# Autodesk Inventor assembly: 090 ASY bottom
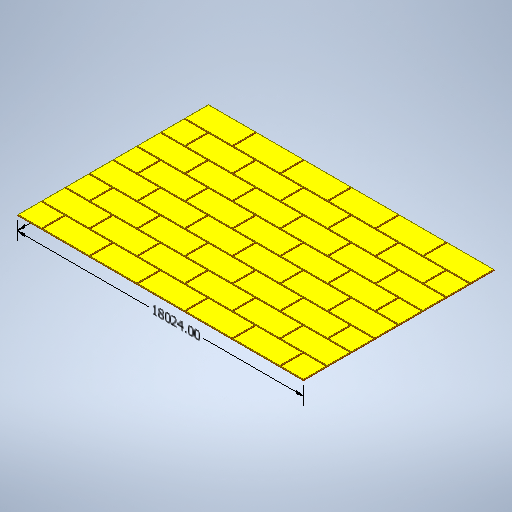
[picture p0: Inventor's stored thumbnail of the model, 512x512]
Saved by Autodesk Inventor 2026.2 (Build 302298000, 298)
## iProperties
Created: 2026-05-19
Part Number: 090 ASY bottom
Document SubType Name: Assembly
Designer: user
Author: user
## Documents named in this file (6)
- C:\Users\admin\Documents\Inventor\GBK-Gubkinskiy\090 ASY bottom.iam
- C:\Users\admin\Documents\Inventor\GBK-Gubkinskiy\0910.ipt
- C:\Users\admin\Documents\Inventor\GBK-Gubkinskiy\092_CPY.iam
- C:\Users\admin\Documents\Inventor\GBK-Gubkinskiy\093_CPY.iam
- C:\Users\admin\Documents\Inventor\GBK-Gubkinskiy\092_CPY1.iam
- C:\Users\admin\Documents\Inventor\GBK-Gubkinskiy\093_CPY1.iam
## Components (53 placed, 5 different names)
1. 0910:1 — Rigid:1
2. 093_CPY:1 [sub-assembly] — Flush:3, Flush:4, Mate:1, Flush:5, Flush:6, Mate:2
3. 093_CPY1:1 [sub-assembly] — Flush:7, Flush:8, Mate:3
4. 093_CPY:2 [sub-assembly]
5. 093_CPY1:2 [sub-assembly]
6. 093_CPY:3 [sub-assembly]
7. 093_CPY1:3 [sub-assembly]
8. 093_CPY:4 [sub-assembly]
9. 093_CPY1:4 [sub-assembly]
10. 092_CPY:1 [sub-assembly] — Rigid:1, Flush:3, Flush:4, Mate:1
11. 092_CPY:2 [sub-assembly]
12. 092_CPY:3 [sub-assembly]
13. 092_CPY:4 [sub-assembly]
14. 092_CPY:5 [sub-assembly]
15. 092_CPY:6 [sub-assembly]
16. 092_CPY:7 [sub-assembly]
17. 092_CPY:8 [sub-assembly]
18. 092_CPY:9 [sub-assembly]
19. 092_CPY:10 [sub-assembly]
20. 092_CPY:11 [sub-assembly]
21. 092_CPY:12 [sub-assembly]
22. 092_CPY:13 [sub-assembly]
23. 092_CPY:14 [sub-assembly]
24. 092_CPY:15 [sub-assembly]
25. 092_CPY:16 [sub-assembly]
26. 092_CPY:17 [sub-assembly]
27. 092_CPY:18 [sub-assembly]
28. 092_CPY:19 [sub-assembly]
29. 092_CPY:20 [sub-assembly]
30. 092_CPY:21 [sub-assembly]
31. 092_CPY:22 [sub-assembly]
32. 092_CPY:23 [sub-assembly]
33. 092_CPY:24 [sub-assembly]
34. 092_CPY1:1 [sub-assembly] — Flush:5, Flush:6, Mate:2
35. 092_CPY1:2 [sub-assembly]
36. 092_CPY1:3 [sub-assembly]
37. 092_CPY1:4 [sub-assembly]
38. 092_CPY1:5 [sub-assembly] — Flush:7, Flush:8, Mate:3
39. 092_CPY1:6 [sub-assembly]
40. 092_CPY1:7 [sub-assembly]
41. 092_CPY1:8 [sub-assembly]
42. 092_CPY1:9 [sub-assembly]
43. 092_CPY1:10 [sub-assembly]
44. 092_CPY1:11 [sub-assembly]
45. 092_CPY1:12 [sub-assembly]
46. 092_CPY1:13 [sub-assembly]
47. 092_CPY1:14 [sub-assembly]
48. 092_CPY1:15 [sub-assembly]
49. 092_CPY1:16 [sub-assembly]
50. 092_CPY1:17 [sub-assembly]
51. 092_CPY1:18 [sub-assembly]
52. 092_CPY1:19 [sub-assembly]
53. 092_CPY1:20 [sub-assembly]
## Component patterns: (4 elements), (4 elements, first: 093_CPY:1 + 093_CPY1:1), (6 elements, first: 092_CPY:1), МассивКомп 1:2 (6 elements), МассивКомп 1:3 (6 elements), МассивКомп 1:4 (6 elements), (5 elements, first: 092_CPY1:1), МассивКомп 2:2 (5 elements), МассивКомп 2:3 (5 elements), МассивКомп 2:4 (5 elements)
## Relationships (10: Flush 6, Mate 3, WeldJoint 1)
- Rigid:1 [WeldJoint] (10 mm): 0910:1 ↔ 092_CPY:1
- Flush:3: 093_CPY:1 ↔ 092_CPY:1
- Flush:4: 093_CPY:1 ↔ 092_CPY:1
- Mate:1 (4 mm): 093_CPY:1 ↔ 092_CPY:1
- Flush:5: 093_CPY:1 ↔ 092_CPY1:1
- Flush:6: 093_CPY:1 ↔ 092_CPY1:1
- Mate:2 (4 mm): 093_CPY:1 ↔ 092_CPY1:1
- Flush:7: 093_CPY1:1 ↔ 092_CPY1:5
- Flush:8: 093_CPY1:1 ↔ 092_CPY1:5
- Mate:3: 093_CPY1:1 ↔ 092_CPY1:5
